# Autodesk Inventor assembly: Jersey_FEA_assembly
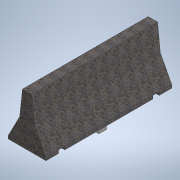
[picture p0: Inventor's stored thumbnail of the model, 180x180]
Saved by Autodesk Inventor 2022 (Build 260153000, 153)
## iProperties
Created: 2021-11-09
Part Number: Jersey_FEA_assembly
Document SubType Name: Assembly
Designer: kibandi
Author: kibandi
## Documents named in this file (9)
- C:\academics\YEAR 4\4.2\DOMS II\DOMS II projects\mechanical design\Jersey_FEA_assembly.iam
- C:\academics\YEAR 4\4.2\DOMS II\DOMS II projects\mechanical design\barrier_pneumatic_connector.ipt
- C:\academics\YEAR 4\4.2\DOMS II\DOMS II projects\mechanical design\Jersey Curb.ipt
- C:\academics\YEAR 4\4.2\DOMS II\DOMS II projects\mechanical design\Jersey_FEA_assembly\AIP\FEA\ds94ji84g.fins
- C:\academics\YEAR 4\4.2\DOMS II\DOMS II projects\mechanical design\Jersey_FEA_assembly\AIP\FEA\ds94ji84g.fsat
- C:\academics\YEAR 4\4.2\DOMS II\DOMS II projects\mechanical design\Jersey_FEA_assembly\AIP\FEA\ds94ji84g.ftes
- C:\academics\YEAR 4\4.2\DOMS II\DOMS II projects\mechanical design\Jersey_FEA_assembly\AIP\FEA\ds94ji84g.fwiz
- C:\academics\YEAR 4\4.2\DOMS II\DOMS II projects\mechanical design\Jersey_FEA_assembly\AIP\FEA\ds94ji874.fmsh
- C:\academics\YEAR 4\4.2\DOMS II\DOMS II projects\mechanical design\Jersey_FEA_assembly\AIP\FEA\ds94ji875.fres
## Components (2 placed, 2 different names)
1. barrier_pneumatic_connector:1 — Mate:2, Mate:4, Mate:7
2. Jersey Curb:1 — Mate:1, Mate:3, Mate:5, Mate:7
## Relationships (7: Mate 7)
- Mate:1: Jersey Curb:1
- Mate:2: barrier_pneumatic_connector:1
- Mate:3: Jersey Curb:1
- Mate:4: barrier_pneumatic_connector:1
- Mate:5: Jersey Curb:1
- Mate:6
- Mate:7: barrier_pneumatic_connector:1 ↔ Jersey Curb:1
## Named parameters: sa_0 = -2.32524e+06, sa_1 = -5.76439e+06, sa_2 = 5e+06
note: some values were not read from the file. Shown as the stored number, unit unknown: "sa_0", "sa_1", "sa_2".
